# Autodesk Inventor assembly: patasTBeam
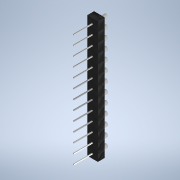
[picture p0: Inventor's stored thumbnail of the model, 180x180]
Saved by Autodesk Inventor 2020 (Build 240168000, 168)
## iProperties
Created: 2022-02-21
Part Number: patasTBeam
Document SubType Name: Assembly
Designer: DANIEL
Author: DANIEL
## Documents named in this file (2)
- C:\Users\DANIEL\Documents\Personal\Convocatorias\Escollera\tesis\CAD\V3\patasTBeam.iam
- C:\Users\DANIEL\Documents\Personal\Convocatorias\Escollera\tesis\CAD\V3\pata.ipt
## Components (13 placed, 1 different names)
1. pata:1 — Coincidencia:1, Coincidencia:2, Coincidencia:3, Coincidencia:29, Coincidencia:30, Coincidencia:32
2. pata:2 — Coincidencia:1, Coincidencia:2, Coincidencia:3, Coincidencia:4, Coincidencia:5, Coincidencia:6
3. pata:3 — Coincidencia:4, Coincidencia:5, Coincidencia:6, Coincidencia:13, Coincidencia:14, Coincidencia:31
4. pata:4 — Coincidencia:13, Coincidencia:14, Coincidencia:31
5. pata:5
6. pata:6 — Coincidencia:34, Coincidencia:35, Coincidencia:36
7. pata:7
8. pata:8
9. pata:9 — Coincidencia:33
10. pata:10 — Coincidencia:33
11. pata:11
12. pata:12 — Coincidencia:29, Coincidencia:30, Coincidencia:32
13. pata:13 — Coincidencia:34, Coincidencia:35, Coincidencia:36
## Relationships (36: Mate 36)
- Coincidencia:1 [Mate]: pata:1 ↔ pata:2
- Coincidencia:2 [Mate]: pata:1 ↔ pata:2
- Coincidencia:3 [Mate]: pata:1 ↔ pata:2
- Coincidencia:4 [Mate]: pata:2 ↔ pata:3
- Coincidencia:5 [Mate]: pata:2 ↔ pata:3
- Coincidencia:6 [Mate]: pata:2 ↔ pata:3
- [Mate]: pata:4 ↔ pata:5
- [Mate]: pata:4 ↔ pata:5
- [Mate]: pata:4 ↔ pata:5
- [Mate]: pata:5 ↔ pata:6
- [Mate]: pata:5 ↔ pata:6
- [Mate]: pata:5 ↔ pata:6
- Coincidencia:13 [Mate]: pata:3 ↔ pata:4
- Coincidencia:14 [Mate]: pata:3 ↔ pata:4
- [Mate]: pata:7 ↔ pata:8
- [Mate]: pata:7 ↔ pata:8
- [Mate]: pata:7 ↔ pata:8
- [Mate]: pata:8 ↔ pata:9
- [Mate]: pata:8 ↔ pata:9
- [Mate]: pata:8 ↔ pata:9
- [Mate]: pata:10 ↔ pata:11
- [Mate]: pata:10 ↔ pata:11
- [Mate]: pata:10 ↔ pata:11
- [Mate]: pata:11 ↔ pata:12
- [Mate]: pata:11 ↔ pata:12
- [Mate]: pata:11 ↔ pata:12
- [Mate]: pata:9 ↔ pata:10
- [Mate]: pata:9 ↔ pata:10
- Coincidencia:29 [Mate]: pata:1 ↔ pata:12
- Coincidencia:30 [Mate]: pata:1 ↔ pata:12
- Coincidencia:31 [Mate]: pata:3 ↔ pata:4
- Coincidencia:32 [Mate]: pata:1 ↔ pata:12
- Coincidencia:33 [Mate]: pata:9 ↔ pata:10
- Coincidencia:34 [Mate]: pata:6 ↔ pata:13
- Coincidencia:35 [Mate]: pata:6 ↔ pata:13
- Coincidencia:36 [Mate]: pata:6 ↔ pata:13
## Named parameters: d6_d0 = 0 mm, d7_d1 = 0 mm, d8_d2 = 0 mm, d9_d3 = 0 mm, d10_d4 = 0 mm, d11_d5 = 0 mm, d14_d0 = 0 mm, d15_d1 = 0 mm, d16_d2 = 0 mm, d17_d3 = 0 mm, d18_d4 = 0 mm, d19_d5 = 0 mm, d20_d6_d0 = 0 mm, d21_d7_d1 = 0 mm, d22_d8_d2 = 0 mm, d23_d9_d3 = 0 mm, d24_d10_d4 = 0 mm, d25_d11_d5 = 0 mm, d26_d12 = 0 mm, d27_d13 = 0 mm
